# Autodesk Inventor assembly: pld-vessel
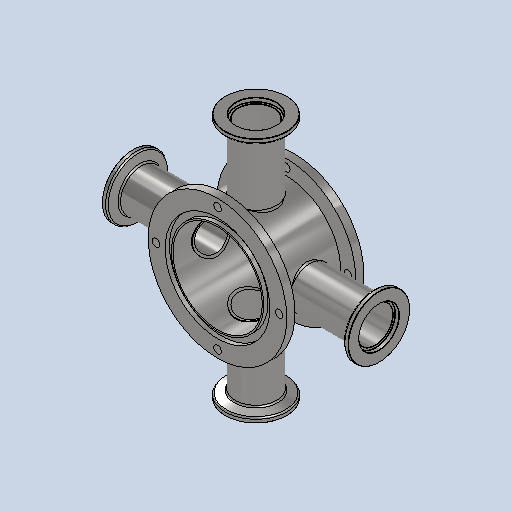
[picture p0: Inventor's stored thumbnail of the model, 512x512]
Saved by Autodesk Inventor 2026 (Build 300175050, 175E)
## iProperties
Created: 2025-11-13
Part Number: pld-vessel
Document SubType Name: Assembly
Designer: kuzmin
Author: kuzmin
## Documents named in this file (3)
- C:\Users\queez\Dropbox\Drawings\PIHTI\PLD\pld-vessel.iam
- C:\Users\queez\Dropbox\Drawings\PIHTI\PLD\pld_vessel.ipt
- C:\Users\queez\Dropbox\Drawings\PIHTI\PLD\pld_vessel_kf_nipple.ipt
## Components (5 placed, 2 different names)
1. pld_vessel:1 — Mate:1, Mate:2, Mate:3
2. pld_vessel_kf_nipple:1
3. pld_vessel_kf_nipple:2
4. pld_vessel_kf_nipple:3
5. pld_vessel_kf_nipple:4
## Relationships (7: WeldJoint 4, Mate 3)
- [WeldJoint]: pld_vessel:1 ↔ pld_vessel_kf_nipple:2
- [WeldJoint]: pld_vessel:1 ↔ pld_vessel_kf_nipple:3
- [WeldJoint]: pld_vessel:1 ↔ pld_vessel_kf_nipple:4
- [WeldJoint]: pld_vessel:1 ↔ pld_vessel_kf_nipple:1
- Mate:1: pld_vessel:1
- Mate:2: pld_vessel:1
- Mate:3: pld_vessel:1
## Named parameters: d0_d2 = 0 mm, d1_d3 = 0 mm
